# Autodesk Inventor assembly: AllAssembled
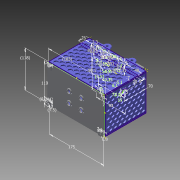
[picture p0: Inventor's stored thumbnail of the model, 180x180]
Saved by Autodesk Inventor 2015 (Build 190159000, 159)
## iProperties
Created: 2015-04-29
Part Number: AllAssembled
Document SubType Name: Assembly
Designer: Akovo_000
Mass: 289.976 g
Surface Area: 3162.49 cm^2
Volume: 281.864 cm^3
Density: 1.02878 g/cm^3
Author: Akovo_000
## Documents named in this file (6)
- C:\Users\Akovo_000\SkyDrive\3D printing\Unibody Enclosure\AllAssembled.iam
- C:\Users\Akovo_000\SkyDrive\3D printing\Unibody Enclosure\Box.ipt
- C:\Users\Akovo_000\SkyDrive\3D printing\Unibody Enclosure\CameraBoardCover.ipt
- C:\Users\Akovo_000\SkyDrive\3D printing\Unibody Enclosure\CIrcutryPLate.ipt
- C:\Users\Akovo_000\SkyDrive\3D printing\Unibody Enclosure\FilterHolder.ipt
- C:\Users\Akovo_000\SkyDrive\3D printing\Unibody Enclosure\SimpleLensPlane.ipt
## Components (5 placed, 5 different names)
1. Box:1 — Rigid:1, Rigid:2
2. CameraBoardCover:1
3. CIrcutryPLate:1 — Rigid:2
4. FilterHolder:1
5. SimpleLensPlane:1 — Rigid:1
## Relationships (2: WeldJoint 2)
- Rigid:1 [WeldJoint] (-3 mm): Box:1 ↔ SimpleLensPlane:1
- Rigid:2 [WeldJoint] (-5 mm): Box:1 ↔ CIrcutryPLate:1
